# Autodesk Inventor assembly: Assembly
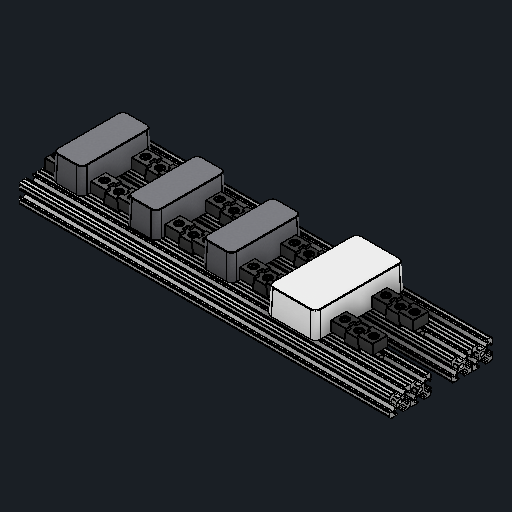
[picture p0: Inventor's stored thumbnail of the model, 512x512]
Saved by Autodesk Inventor 2026.2 (Build 302298000, 298)
## iProperties
Created: 2026-05-18
Part Number: Assembly
Document SubType Name: Assembly
Designer: JoshuaEah
Author: JoshuaEah
## Documents named in this file (7)
- C:\Users\JoshuaEah\Documents\GitHub\Designed-Trinkets\Modular Pedalboard\Assembly.iam
- C:\Users\JoshuaEah\Documents\GitHub\Designed-Trinkets\Modular Pedalboard\1x1 Alu Extrusion.ipt
- 1x1" Alu Extrusion.ipt
- C:\Users\JoshuaEah\Documents\GitHub\Designed-Trinkets\Modular Pedalboard\Compressor.ipt
- C:\Users\JoshuaEah\Documents\GitHub\Designed-Trinkets\Modular Pedalboard\Drive.ipt
- C:\Users\JoshuaEah\Documents\GitHub\Designed-Trinkets\Modular Pedalboard\2-Way Assembly.iam
- C:\Users\JoshuaEah\Documents\GitHub\Designed-Trinkets\Modular Pedalboard\Endstop Assembly.iam
## Components (18 placed, 5 different names)
1. 1x1 Alu Extrusion:1 — Flush:1, Flush:2, Flush:3, Flush:4, Mate:12, Mate:15, Mate:27, Mate:28, Mate:29, Mate:30
2. 1x1 Alu Extrusion:2 — Flush:1, Flush:4, Flush:5, Mate:12, Mate:13, Planar:1, Planar:2, Planar:5, Mate:33, Mate:35, Planar:7, Planar:9, Mate:37
3. 1x1 Alu Extrusion:3 — Flush:2, Flush:5, Flush:6, Mate:13, Mate:14, Planar:3, Planar:4, Mate:31, Mate:32, Planar:6, Mate:34, Planar:8, Mate:36, Planar:10, Mate:40
4. 1x1 Alu Extrusion:4 — Flush:3, Flush:6, Mate:14
5. Compressor:1 — Mate:15
6. Drive:1 — Mate:27
7. Drive:2 — Mate:28
8. Drive:3 — Mate:29
9. 2-Way Assembly:1 [sub-assembly] — Planar:1
10. 2-Way Assembly:2 [sub-assembly] — Planar:2, Mate:30
11. 2-Way Assembly:3 [sub-assembly] — Planar:3, Mate:31
12. 2-Way Assembly:4 [sub-assembly] — Planar:4, Mate:32
13. 2-Way Assembly:5 [sub-assembly] — Planar:5, Mate:33
14. 2-Way Assembly:6 [sub-assembly] — Planar:6, Mate:34
15. 2-Way Assembly:7 [sub-assembly] — Mate:35, Planar:7
16. 2-Way Assembly:8 [sub-assembly] — Planar:8, Mate:36
17. Endstop Assembly:1 [sub-assembly] — Planar:9, Mate:37
18. Endstop Assembly:2 [sub-assembly] — Planar:10, Mate:40
## Relationships (34: Mate 18, PlanarJoint 10, Flush 6)
- Planar:1: 1x1 Alu Extrusion:2 ↔ 2-Way Assembly:1
- [Mate]: 1x1 Alu Extrusion:1 ↔ 2-Way Assembly:1
- Flush:1: 1x1 Alu Extrusion:1 ↔ 1x1 Alu Extrusion:2
- Flush:2: 1x1 Alu Extrusion:1 ↔ 1x1 Alu Extrusion:3
- Flush:3: 1x1 Alu Extrusion:1 ↔ 1x1 Alu Extrusion:4
- Flush:4: 1x1 Alu Extrusion:1 ↔ 1x1 Alu Extrusion:2
- Flush:5: 1x1 Alu Extrusion:2 ↔ 1x1 Alu Extrusion:3
- Flush:6: 1x1 Alu Extrusion:3 ↔ 1x1 Alu Extrusion:4
- Mate:12: 1x1 Alu Extrusion:1 ↔ 1x1 Alu Extrusion:2
- Mate:13 (25.4 mm): 1x1 Alu Extrusion:2 ↔ 1x1 Alu Extrusion:3
- Mate:14: 1x1 Alu Extrusion:3 ↔ 1x1 Alu Extrusion:4
- Mate:15: 1x1 Alu Extrusion:1 ↔ Compressor:1
- Mate:27: 1x1 Alu Extrusion:1 ↔ Drive:1
- Mate:28: 1x1 Alu Extrusion:1 ↔ Drive:2
- Mate:29: 1x1 Alu Extrusion:1 ↔ Drive:3
- Planar:2: 1x1 Alu Extrusion:2 ↔ 2-Way Assembly:2
- Mate:30: 1x1 Alu Extrusion:1 ↔ 2-Way Assembly:2
- Planar:3: 1x1 Alu Extrusion:3 ↔ 2-Way Assembly:3
- Planar:4: 1x1 Alu Extrusion:3 ↔ 2-Way Assembly:4
- Mate:31: 1x1 Alu Extrusion:3 ↔ 2-Way Assembly:3
- Mate:32: 1x1 Alu Extrusion:3 ↔ 2-Way Assembly:4
- Planar:5: 1x1 Alu Extrusion:2 ↔ 2-Way Assembly:5
- Mate:33: 1x1 Alu Extrusion:2 ↔ 2-Way Assembly:5
- Planar:6: 1x1 Alu Extrusion:3 ↔ 2-Way Assembly:6
- Mate:34: 1x1 Alu Extrusion:3 ↔ 2-Way Assembly:6
- Mate:35: 1x1 Alu Extrusion:2 ↔ 2-Way Assembly:7
- Planar:7: 1x1 Alu Extrusion:2 ↔ 2-Way Assembly:7
- Planar:8: 1x1 Alu Extrusion:3 ↔ 2-Way Assembly:8
- Mate:36: 1x1 Alu Extrusion:3 ↔ 2-Way Assembly:8
- Planar:9: 1x1 Alu Extrusion:2 ↔ Endstop Assembly:1
- Mate:37: 1x1 Alu Extrusion:2 ↔ Endstop Assembly:1
- [Mate]: 1x1 Alu Extrusion:2 ↔ Endstop Assembly:1
- Planar:10: 1x1 Alu Extrusion:3 ↔ Endstop Assembly:2
- Mate:40: 1x1 Alu Extrusion:3 ↔ Endstop Assembly:2
